# Autodesk Inventor assembly: KB33-046-003 - Модуль мотора в сборе
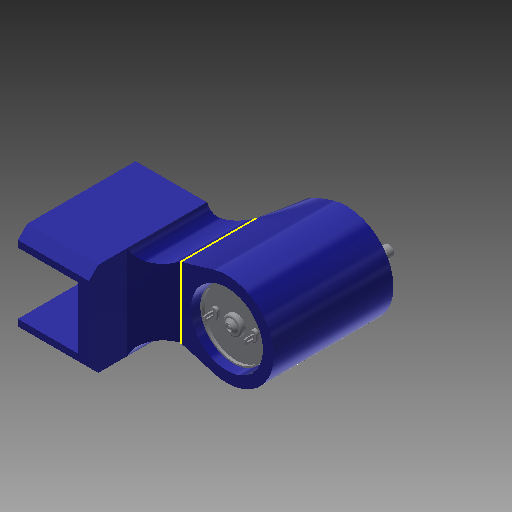
[picture p0: Inventor's stored thumbnail of the model, 512x512]
Saved by Autodesk Inventor 2019 (Build 230136000, 136)
## iProperties
Created: 2021-06-09
Part Number: KB33-046-003 - Модуль мотора в сборе
Material: Типовые
Document SubType Name: Assembly
Designer: Петров Иван
Author: Петров Иван
## Documents named in this file (3)
- E:\IVAN\Ivan_desktop\Kvantorium\Projects\RoboPatrol\design\KB33-046-003 - Модуль мотора в сборе.iam
- E:\IVAN\Ivan_desktop\Kvantorium\Projects\RoboPatrol\design\KB33-046-003-001 - Крепление.ipt
- E:\IVAN\Ivan_desktop\Kvantorium\Projects\RoboPatrol\design\standart_components\dc_gear_motor_12V_500rpm\dc_gear_motor_12V_500rpm.ipt
## Components (2 placed, 2 different names)
1. KB33-046-003-001 - Крепление:1 — Mate:1, Mate:2, Mate:3
2. dc_gear_motor_12V_500rpm:1 — Mate:1, Mate:2, Mate:3
## Relationships (3: Mate 3)
- Mate:1: KB33-046-003-001 - Крепление:1 ↔ dc_gear_motor_12V_500rpm:1
- Mate:2: KB33-046-003-001 - Крепление:1 ↔ dc_gear_motor_12V_500rpm:1
- Mate:3: KB33-046-003-001 - Крепление:1 ↔ dc_gear_motor_12V_500rpm:1
